# Autodesk Inventor assembly: full guns
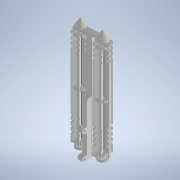
[picture p0: Inventor's stored thumbnail of the model, 180x180]
Saved by Autodesk Inventor 2020.1 (Build 241239000, 239)
## iProperties
Created: 2022-03-19
Part Number: full guns
Document SubType Name: Assembly
Designer: User
Author: User
## Documents named in this file (7)
- D:\GitHub\TANK\3D-turret\full guns.iam
- D:\GitHub\TANK\3D-turret\gun.iam
- D:\GitHub\TANK\3D-turret\соединение пушек.ipt
- D:\GitHub\TANK\3D-turret\подшипник.ipt
- D:\GitHub\TANK\3D-turret\центр пушки.ipt
- D:\GitHub\TANK\3D-turret\держак середины пушки.ipt
- D:\GitHub\TANK\3D-turret\соединение пушек перед.ipt
## Components (10 placed, 6 different names)
1. gun:2 [sub-assembly] — С поворотом:1
2. gun:3 [sub-assembly] — С поворотом:2
3. подшипник:1 — С поворотом:2, Жесткий:9
4. подшипник:2 — С поворотом:1, Жесткий:10
5. центр пушки:1 — Жесткий:6, Жесткий:7, Жесткий:8
6. соединение пушек:2 — Жесткий:6
7. подшипник:3
8. подшипник:4
9. держак середины пушки:1 — Жесткий:7
10. соединение пушек перед:1 — Жесткий:8, Жесткий:9, Жесткий:10
## Relationships (9: WeldJoint 7, RevoluteJoint 2)
- С поворотом:1 [RevoluteJoint]: gun:2 ↔ подшипник:2
- С поворотом:2 [RevoluteJoint]: gun:3 ↔ подшипник:1
- [WeldJoint]: соединение пушек:2 ↔ подшипник:3
- [WeldJoint]: соединение пушек:2 ↔ подшипник:4
- Жесткий:6 [WeldJoint]: центр пушки:1 ↔ соединение пушек:2
- Жесткий:7 [WeldJoint]: центр пушки:1 ↔ держак середины пушки:1
- Жесткий:8 [WeldJoint]: центр пушки:1 ↔ соединение пушек перед:1
- Жесткий:9 [WeldJoint]: подшипник:1 ↔ соединение пушек перед:1
- Жесткий:10 [WeldJoint]: подшипник:2 ↔ соединение пушек перед:1
## Named parameters: d10_d0 = 0 mm, d11_d1 = 0 mm
